# Autodesk Inventor assembly: elric20
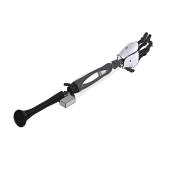
[picture p0: Inventor's stored thumbnail of the model, 180x180]
Saved by Autodesk Inventor 2020.2 (Build 242310000, 310)
## iProperties
Created: 2020-04-12
Part Number: elric20
Document SubType Name: Assembly
Designer: Bardo91
Author: Bardo91
## Documents named in this file (3)
- D:\programming\elric\hardware\elric20.iam
- D:\programming\elric\hardware\1. hand\elric20-01A.iam
- D:\programming\elric\hardware\2. arm\elric20-02A.iam
## Components (2 placed, 2 different names)
1. elric20-01A:1 [sub-assembly] — Mate:1, Mate:2
2. elric20-02A:1 [sub-assembly] — Mate:1, Mate:2
## Relationships (2: Mate 2)
- Mate:1: elric20-01A:1 ↔ elric20-02A:1
- Mate:2 (0.5 mm): elric20-01A:1 ↔ elric20-02A:1
